# Autodesk Inventor assembly: Assembly
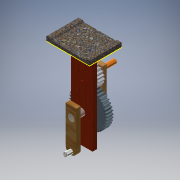
[picture p0: Inventor's stored thumbnail of the model, 180x180]
Saved by Autodesk Inventor 2016 (Build 200138000, 138)
## iProperties
Created: 2015-10-29
Part Number: Assembly
Document SubType Name: Assembly
Designer: Meet
Author: Meet
## Documents named in this file (10)
- C:\Users\Meet\Documents\College\Study Material\EG\EG Autodesk Drawings\meet\Assembly.iam
- C:\Users\Meet\Documents\College\Study Material\EG\EG Autodesk Drawings\meet\base.ipt
- C:\Users\Meet\Documents\College\Study Material\EG\EG Autodesk Drawings\meet\column.ipt
- C:\Users\Meet\Documents\College\Study Material\EG\EG Autodesk Drawings\meet\driven_shaft.ipt
- C:\Users\Meet\Documents\College\Study Material\EG\EG Autodesk Drawings\meet\driving_shaft.ipt
- C:\Users\Meet\Documents\College\Study Material\EG\EG Autodesk Drawings\meet\gear_big.ipt
- C:\Users\Meet\Documents\College\Study Material\EG\EG Autodesk Drawings\meet\gear_small.ipt
- C:\Users\Meet\Documents\College\Study Material\EG\EG Autodesk Drawings\meet\handle_crank.ipt
- C:\Users\Meet\Documents\College\Study Material\EG\EG Autodesk Drawings\meet\handle.ipt
- C:\Users\Meet\Documents\College\Study Material\EG\EG Autodesk Drawings\meet\crank.ipt
## Components (9 placed, 9 different names)
1. base:1 — Mate:1, Flush:1, Flush:2, Flush:3
2. column:1 — Mate:1, Flush:1, Flush:2, Insert:1, Insert:2, Flush:3, Angle:2
3. driven_shaft:1 — Insert:1, Insert:4, Insert:8
4. driving_shaft:1 — Insert:2, Insert:3, Insert:5, Insert:7, Flush:4
5. gear_big:1 — Insert:3, Rotation:2, Flush:4, Angle:1
6. gear_small:1 — Insert:4, Rotation:2
7. handle_crank:1 — Insert:5, Angle:1, Insert:9, Angle:2
8. crank:1 — Insert:7, Insert:8
9. handle:1 — Insert:9
## Relationships (16: Insert 8, Flush 4, Angle 2, Mate 1, RelateRotation 1)
- Mate:1: base:1 ↔ column:1
- Flush:1 (25 mm): base:1 ↔ column:1
- Flush:2 (32.5 mm): base:1 ↔ column:1
- Insert:1: column:1 ↔ driven_shaft:1
- Insert:2: column:1 ↔ driving_shaft:1
- Insert:3: driving_shaft:1 ↔ gear_big:1
- Insert:4: driven_shaft:1 ↔ gear_small:1
- Flush:3 (25 mm): base:1 ↔ column:1
- Insert:5: driving_shaft:1 ↔ handle_crank:1
- Insert:7: driving_shaft:1 ↔ crank:1
- Insert:8 (0.5 mm): driven_shaft:1 ↔ crank:1
- Rotation:2 [RelateRotation] (2 ul): gear_big:1 ↔ gear_small:1
- Flush:4: driving_shaft:1 ↔ gear_big:1
- Angle:1 (0 deg): gear_big:1 ↔ handle_crank:1
- Insert:9: handle_crank:1 ↔ handle:1
- Angle:2 (360 deg): column:1 ↔ handle_crank:1
